# Autodesk Inventor assembly: DensGlass
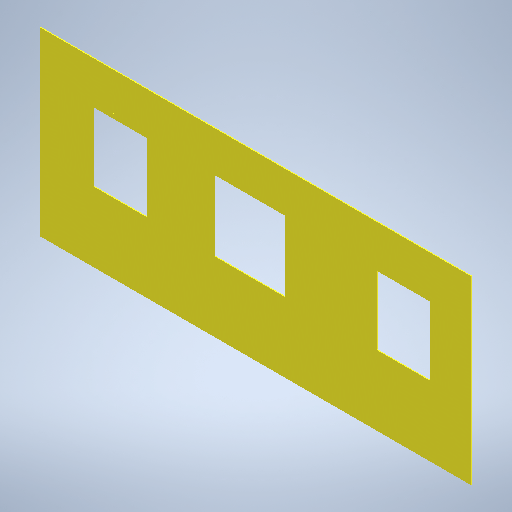
[picture p0: Inventor's stored thumbnail of the model, 512x512]
Saved by Autodesk Inventor 2025.1 (Build 291241020, 241B)
## iProperties
Created: 2024-10-03
Part Number: DensGlass
Document SubType Name: Assembly
Designer: Tom
Author: Tom
## Documents named in this file (7)
- C:\Users\Tom\Documents\Inventor\Mobility\Additional_Building\DensGlass.iam
- C:\Users\Tom\Documents\Inventor\Mobility\Additional_Building\DensGlass_With_Dimensions_12_x_60.6875_Inches.ipt
- C:\Users\Tom\Documents\Inventor\Mobility\Additional_Building\DensGlass_With_Dimensions_36.5_x_48_Inches.ipt
- C:\Users\Tom\Documents\Inventor\Mobility\Additional_Building\DensGlass_With_Dimensions_48_x_96_Inches.ipt
- C:\Users\Tom\Documents\Inventor\Mobility\Additional_Building\DensGlass_With_Dimensions_48_x_84.5_Inches.ipt
- C:\Users\Tom\Documents\Inventor\Mobility\Additional_Building\DensGlass_With_Dimensions_25.375_x_36.5_Inches.ipt
- C:\Users\Tom\Documents\Inventor\Mobility\Additional_Building\DensGlass_With_Dimensions_25.375_x_96_Inches.ipt
## Components (15 placed, 6 different names)
1. DensGlass_With_Dimensions_48_x_96_Inches:3 — Mate:5, Mate:6, Flush:6
2. DensGlass_With_Dimensions_48_x_96_Inches:1 — Flush:3, Mate:2, Flush:4, Mate:5
3. DensGlass_With_Dimensions_48_x_96_Inches:2
4. DensGlass_With_Dimensions_36.5_x_48_Inches:1 — Mate:1, Flush:1, Flush:2, Flush:3, Mate:2, Flush:4, Mate:3, Flush:5
5. DensGlass_With_Dimensions_36.5_x_48_Inches:2
6. DensGlass_With_Dimensions_12_x_60.6875_Inches:1 — Mate:1, Flush:1, Flush:2, Mate:4
7. DensGlass_With_Dimensions_12_x_60.6875_Inches:2 — Mate:8
8. DensGlass_With_Dimensions_12_x_60.6875_Inches:3
9. DensGlass_With_Dimensions_12_x_60.6875_Inches:4
10. DensGlass_With_Dimensions_48_x_84.5_Inches:1 — Mate:3, Mate:4, Flush:5, Mate:6, Flush:6, Mate:7, Flush:7, Mate:9
11. DensGlass_With_Dimensions_48_x_84.5_Inches:2
12. DensGlass_With_Dimensions_25.375_x_96_Inches:1 — Mate:9, Mate:10, Flush:8
13. DensGlass_With_Dimensions_25.375_x_96_Inches:2
14. DensGlass_With_Dimensions_25.375_x_36.5_Inches:1 — Mate:7, Mate:8, Flush:7, Mate:10, Flush:8
15. DensGlass_With_Dimensions_25.375_x_36.5_Inches:2
## Component patterns: (2 elements, first: DensGlass_With_Dimensions_48_x_96_Inches:1), (2 elements, first: DensGlass_With_Dimensions_36.5_x_48_Inches:1), (4 elements, first: DensGlass_With_Dimensions_12_x_60.6875_Inches:1), (2 elements, first: DensGlass_With_Dimensions_48_x_84.5_Inches:1), (2 elements, first: DensGlass_With_Dimensions_25.375_x_96_Inches:1), (2 elements, first: DensGlass_With_Dimensions_25.375_x_36.5_Inches:1)
## Relationships (18: Mate 10, Flush 8)
- Mate:1: DensGlass_With_Dimensions_36.5_x_48_Inches:1 ↔ DensGlass_With_Dimensions_12_x_60.6875_Inches:1
- Flush:1: DensGlass_With_Dimensions_36.5_x_48_Inches:1 ↔ DensGlass_With_Dimensions_12_x_60.6875_Inches:1
- Flush:2: DensGlass_With_Dimensions_36.5_x_48_Inches:1 ↔ DensGlass_With_Dimensions_12_x_60.6875_Inches:1
- Flush:3: DensGlass_With_Dimensions_48_x_96_Inches:1 ↔ DensGlass_With_Dimensions_36.5_x_48_Inches:1
- Mate:2: DensGlass_With_Dimensions_48_x_96_Inches:1 ↔ DensGlass_With_Dimensions_36.5_x_48_Inches:1
- Flush:4: DensGlass_With_Dimensions_48_x_96_Inches:1 ↔ DensGlass_With_Dimensions_36.5_x_48_Inches:1
- Mate:3: DensGlass_With_Dimensions_36.5_x_48_Inches:1 ↔ DensGlass_With_Dimensions_48_x_84.5_Inches:1
- Mate:4: DensGlass_With_Dimensions_12_x_60.6875_Inches:1 ↔ DensGlass_With_Dimensions_48_x_84.5_Inches:1
- Flush:5: DensGlass_With_Dimensions_36.5_x_48_Inches:1 ↔ DensGlass_With_Dimensions_48_x_84.5_Inches:1
- Mate:5: DensGlass_With_Dimensions_48_x_96_Inches:3 ↔ DensGlass_With_Dimensions_48_x_96_Inches:1
- Mate:6: DensGlass_With_Dimensions_48_x_96_Inches:3 ↔ DensGlass_With_Dimensions_48_x_84.5_Inches:1
- Flush:6: DensGlass_With_Dimensions_48_x_96_Inches:3 ↔ DensGlass_With_Dimensions_48_x_84.5_Inches:1
- Mate:7: DensGlass_With_Dimensions_48_x_84.5_Inches:1 ↔ DensGlass_With_Dimensions_25.375_x_36.5_Inches:1
- Mate:8: DensGlass_With_Dimensions_12_x_60.6875_Inches:2 ↔ DensGlass_With_Dimensions_25.375_x_36.5_Inches:1
- Flush:7: DensGlass_With_Dimensions_48_x_84.5_Inches:1 ↔ DensGlass_With_Dimensions_25.375_x_36.5_Inches:1
- Mate:9: DensGlass_With_Dimensions_48_x_84.5_Inches:1 ↔ DensGlass_With_Dimensions_25.375_x_96_Inches:1
- Mate:10: DensGlass_With_Dimensions_25.375_x_96_Inches:1 ↔ DensGlass_With_Dimensions_25.375_x_36.5_Inches:1
- Flush:8: DensGlass_With_Dimensions_25.375_x_96_Inches:1 ↔ DensGlass_With_Dimensions_25.375_x_36.5_Inches:1
